# Autodesk Inventor assembly: 4.25'' diameter Turntable Bearing
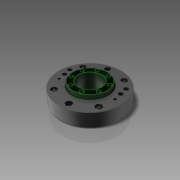
[picture p0: Inventor's stored thumbnail of the model, 180x180]
Saved by Autodesk Inventor 2012 (Build 160160000, 160)
## iProperties
Created: 2011-04-20
Part Number: 4.25'' diameter Turntable Bearing
Document SubType Name: Assembly
Designer: Jordan
Mass: 100.893 g
Surface Area: 959.867 cm^2
Volume: 81.1309 cm^3
Density: 1.24358 g/cm^3
Translation Standard: STEP AP203
FileName: 276-1810-LARGE.STEP
PreProcessor: SolidWorks 2010
PostProcessor: Build: 160, Release: 2012 RTM - Date: Tue 03/01/2011
Sent Units: inch
Uncertainty: 1e-05
Author: Jordan
## Documents named in this file (6)
- C:\Users\Jordan\Documents\VEX CAD Parts\Gears & Pulleys\(66-Tooth) 4.25'' diameter Turntable Bearing.iam
- C:\Users\Jordan\Documents\VEX CAD Parts\Gears & Pulleys\(66-Tooth) 4.25'' diameter Turntable Bearing-Parts\66-Tooth Spur Gear.ipt
- C:\Users\Jordan\Documents\VEX CAD Parts\Gears & Pulleys\(66-Tooth) 4.25'' diameter Turntable Bearing-Parts\Bottom.ipt
- C:\Users\Jordan\Documents\VEX CAD Parts\Gears & Pulleys\(66-Tooth) 4.25'' diameter Turntable Bearing-Parts\Top.ipt
- C:\Users\Jordan\Documents\VEX CAD Parts\Screws & Nuts\Nut 8-32 Nylock.ipt
- C:\Users\Jordan\Documents\VEX CAD Parts\Screws & Nuts\Screw 8-32 x 0.750''-Silver.ipt
## Components (11 placed, 5 different names)
1. Nut 8-32 Nylock:1 — Mate:20, Mate:21
2. Nut 8-32 Nylock:2 — Mate:15, Mate:16
3. 66-Tooth Spur Gear:1 — Mate:22, Mate:23, Mate:24
4. Screw 8-32 x 0.750''-Silver:1 — Mate:7, Mate:8, Mate:9, Mate:11
5. Screw 8-32 x 0.750''-Silver:2 — Mate:12, Mate:13, Mate:14, Mate:16
6. Bottom:1 — Mate:1, Mate:2, Mate:6, Mate:7, Mate:8, Mate:12, Mate:13, Mate:17, Mate:18, Mate:23, Mate:24
7. Nut 8-32 Nylock:3 — Mate:3, Mate:4
8. Screw 8-32 x 0.750''-Silver:3 — Mate:1, Mate:2, Mate:4, Mate:5
9. Screw 8-32 x 0.750''-Silver:4 — Mate:17, Mate:18, Mate:19, Mate:21
10. Top:1 — Mate:3, Mate:5, Mate:6, Mate:9, Mate:10, Mate:14, Mate:15, Mate:19, Mate:20, Mate:22
11. Nut 8-32 Nylock:4 — Mate:10, Mate:11
## Relationships (24: Mate 24)
- Mate:1: Bottom:1 ↔ Screw 8-32 x 0.750''-Silver:3
- Mate:2: Bottom:1 ↔ Screw 8-32 x 0.750''-Silver:3
- Mate:3: Nut 8-32 Nylock:3 ↔ Top:1
- Mate:4: Nut 8-32 Nylock:3 ↔ Screw 8-32 x 0.750''-Silver:3
- Mate:5: Screw 8-32 x 0.750''-Silver:3 ↔ Top:1
- Mate:6: Bottom:1 ↔ Top:1
- Mate:7: Screw 8-32 x 0.750''-Silver:1 ↔ Bottom:1
- Mate:8: Screw 8-32 x 0.750''-Silver:1 ↔ Bottom:1
- Mate:9: Screw 8-32 x 0.750''-Silver:1 ↔ Top:1
- Mate:10: Top:1 ↔ Nut 8-32 Nylock:4
- Mate:11: Screw 8-32 x 0.750''-Silver:1 ↔ Nut 8-32 Nylock:4
- Mate:12: Screw 8-32 x 0.750''-Silver:2 ↔ Bottom:1
- Mate:13: Screw 8-32 x 0.750''-Silver:2 ↔ Bottom:1
- Mate:14: Screw 8-32 x 0.750''-Silver:2 ↔ Top:1
- Mate:15: Nut 8-32 Nylock:2 ↔ Top:1
- Mate:16: Nut 8-32 Nylock:2 ↔ Screw 8-32 x 0.750''-Silver:2
- Mate:17: Bottom:1 ↔ Screw 8-32 x 0.750''-Silver:4
- Mate:18: Bottom:1 ↔ Screw 8-32 x 0.750''-Silver:4
- Mate:19: Screw 8-32 x 0.750''-Silver:4 ↔ Top:1
- Mate:20: Nut 8-32 Nylock:1 ↔ Top:1
- Mate:21: Nut 8-32 Nylock:1 ↔ Screw 8-32 x 0.750''-Silver:4
- Mate:22: 66-Tooth Spur Gear:1 ↔ Top:1
- Mate:23: 66-Tooth Spur Gear:1 ↔ Bottom:1
- Mate:24: 66-Tooth Spur Gear:1 ↔ Bottom:1
